# Autodesk Inventor assembly: Ensemble tout
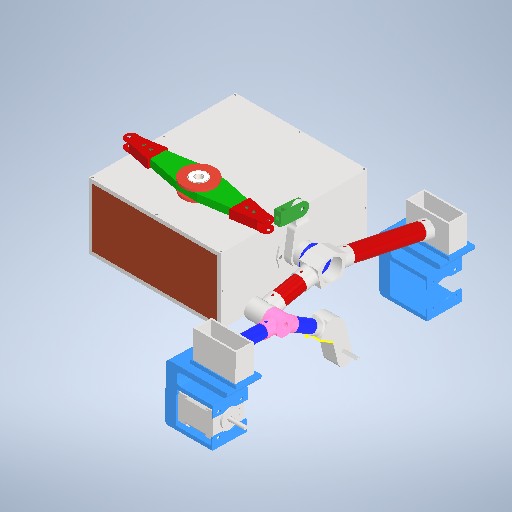
[picture p0: Inventor's stored thumbnail of the model, 512x512]
Saved by Autodesk Inventor 2026.2 (Build 302298010, 298A)
## iProperties
Created: 2026-03-16
Part Number: Ensemble tout
Document SubType Name: Assembly
Designer: genon
Author: genon
## Documents named in this file (20)
- C:\Users\genon\Documents\Henallux Passerelle\Projet de conception\Cassini T-X\Inventor\Ensemble tout.iam
- C:\Users\genon\Documents\Henallux Passerelle\Projet de conception\Cassini T-X\Inventor\Ensemble_Boite_chassis.iam
- C:\Users\genon\Documents\Henallux Passerelle\Projet de conception\Cassini T-X\Inventor\Suspension\Ensemble_Relier_suspension.iam
- C:\Users\genon\Documents\Henallux Passerelle\Projet de conception\Cassini T-X\Inventor\Suspension\tube vers bogie.ipt
- C:\Users\genon\Documents\Henallux Passerelle\Projet de conception\Cassini T-X\Inventor\Suspension\bielle sup.ipt
- C:\Users\genon\Documents\Henallux Passerelle\Projet de conception\Cassini T-X\Inventor\Suspension\bielle côté 0.ipt
- C:\Users\genon\Documents\Henallux Passerelle\Projet de conception\Cassini T-X\Inventor\Suspension\bièlle côté.ipt
- C:\Users\genon\Documents\Henallux Passerelle\Projet de conception\Cassini T-X\Inventor\Suspension\Rolling v2.ipt
- C:\Users\genon\Documents\Henallux Passerelle\Projet de conception\Cassini T-X\Inventor\Suspension\bielle côté 2.ipt
- C:\Users\genon\Documents\Henallux Passerelle\Projet de conception\Cassini T-X\Inventor\Suspension\bielle côté 3.ipt
- C:\Users\genon\Documents\Henallux Passerelle\Projet de conception\Cassini T-X\Inventor\Suspension\tubelong_rocker.ipt
- C:\Users\genon\Documents\Henallux Passerelle\Projet de conception\Cassini T-X\Inventor\Suspension\Attache servomoteur.ipt
- C:\Users\genon\Documents\Henallux Passerelle\Projet de conception\Cassini T-X\Inventor\Suspension\Attache moteur.ipt
- C:\Users\genon\Documents\Henallux Passerelle\Projet de conception\Cassini T-X\Inventor\Suspension\bielle rocker.ipt
- C:\Users\genon\Documents\Henallux Passerelle\Projet de conception\Cassini T-X\Inventor\Suspension\bielle rocker2.ipt
- C:\Users\genon\Documents\Henallux Passerelle\Projet de conception\Cassini T-X\Inventor\Suspension\tube des bogies.ipt
- C:\Users\genon\Documents\Henallux Passerelle\Projet de conception\Cassini T-X\Inventor\Suspension\bielle roue milieu.ipt
- C:\Users\genon\Documents\Henallux Passerelle\Projet de conception\Cassini T-X\Inventor\Suspension\Attache servomoteur_bogie.ipt
- C:\Users\genon\Documents\Henallux Passerelle\Projet de conception\Cassini T-X\Inventor\Suspension\mr_105_2rs.ipt
- C:\Users\genon\Downloads\nema17_17hs19-2004s1_stepperonline-1.snapshot.1\NEMA17_17HS19-2004S1_Stepperonline\NEMA17_17HS19-2004S1_Stepperonline\NEMA17_17HS19-2004S1_Stepperonline.ipt
## Components (23 placed, 19 different names)
1. Ensemble_Boite_chassis:1 [sub-assembly] — Placage:1, Placage:2, Placage:15, Placage:16, Placage:17
2. Ensemble_Relier_suspension:1 [sub-assembly] — Placage:1, Placage:2
3. bielle sup:1 — Placage:53, Placage:54
4. bielle côté 0:1 — Placage:15, Placage:16, Placage:17, Cylindrique:2, Placage:19
5. bièlle côté:1 — Cylindrique:1, Placage:18, Placage:19, Placage:20, Placage:21, Placage:22, Cylindrique:3, Cylindrique:6, Placage:52, Placage:54
6. Rolling v2:1 — Cylindrique:1, Placage:18, Cylindrique:2
7. bielle côté 2:1 — Placage:20, Placage:21, Placage:22, Placage:23, Placage:24, Placage:25, Placage:26, Placage:27
8. Rolling v2:2 — Cylindrique:3, Placage:23
9. bielle côté 3:1 — Placage:24, Placage:25, Placage:26, Placage:27, Placage:28, Placage:29, Placage:35, Placage:36
10. tubelong_rocker:1 — Placage:28, Placage:29, Placage:30, Placage:31
11. Attache servomoteur:1 — Placage:30, Placage:31, Placage:32, Placage:33, Placage:34
12. Attache moteur:2 — Placage:32, Placage:33, Placage:34
13. tube vers bogie:3 — Placage:35, Placage:36, Placage:37, Placage:38
14. bielle rocker:1 — Placage:37, Placage:38, Cylindrique:4, Placage:39, Placage:40
15. Rolling v2:3 — Cylindrique:4, Placage:39, Cylindrique:5
16. bielle rocker2:1 — Placage:40, Cylindrique:5, Placage:41, Placage:42, Placage:43, Placage:44
17. tube des bogies:1 — Placage:43, Placage:44, Placage:47, Placage:48
18. tube des bogies:2 — Placage:41, Placage:42, Placage:45, Placage:46
19. bielle roue milieu:1 — Placage:45, Placage:46
20. Attache servomoteur_bogie:1 — Placage:47, Placage:48, Placage:49, Placage:50, Placage:51
21. Attache moteur:3 — Placage:49, Placage:50, Placage:51, Placage:55, Placage:56, Placage:57
22. mr_105_2rs:1 — Cylindrique:6, Placage:52, Placage:53
23. NEMA17_17HS19-2004S1_Stepperonline:1 — Placage:55, Placage:56, Placage:57
## Relationships (51: Mate 45, CylindricalJoint 6)
- Placage:1 [Mate]: Ensemble_Boite_chassis:1 ↔ Ensemble_Relier_suspension:1
- Placage:2 [Mate]: Ensemble_Boite_chassis:1 ↔ Ensemble_Relier_suspension:1
- Placage:15 [Mate]: Ensemble_Boite_chassis:1 ↔ bielle côté 0:1
- Placage:16 [Mate]: Ensemble_Boite_chassis:1 ↔ bielle côté 0:1
- Placage:17 [Mate]: Ensemble_Boite_chassis:1 ↔ bielle côté 0:1
- Cylindrique:1: bièlle côté:1 ↔ Rolling v2:1
- Placage:18 [Mate]: bièlle côté:1 ↔ Rolling v2:1
- Cylindrique:2: bielle côté 0:1 ↔ Rolling v2:1
- Placage:19 [Mate]: bielle côté 0:1 ↔ bièlle côté:1
- Placage:20 [Mate]: bièlle côté:1 ↔ bielle côté 2:1
- Placage:21 [Mate]: bièlle côté:1 ↔ bielle côté 2:1
- Placage:22 [Mate]: bièlle côté:1 ↔ bielle côté 2:1
- Cylindrique:3: bièlle côté:1 ↔ Rolling v2:2
- Placage:23 [Mate]: bielle côté 2:1 ↔ Rolling v2:2
- Placage:24 [Mate]: bielle côté 2:1 ↔ bielle côté 3:1
- Placage:25 [Mate]: bielle côté 2:1 ↔ bielle côté 3:1
- Placage:26 [Mate]: bielle côté 2:1 ↔ bielle côté 3:1
- Placage:27 [Mate]: bielle côté 2:1 ↔ bielle côté 3:1
- Placage:28 [Mate]: bielle côté 3:1 ↔ tubelong_rocker:1
- Placage:29 [Mate]: bielle côté 3:1 ↔ tubelong_rocker:1
- Placage:30 [Mate]: tubelong_rocker:1 ↔ Attache servomoteur:1
- Placage:31 [Mate]: tubelong_rocker:1 ↔ Attache servomoteur:1
- Placage:32 [Mate]: Attache servomoteur:1 ↔ Attache moteur:2
- Placage:33 [Mate]: Attache servomoteur:1 ↔ Attache moteur:2
- Placage:34 [Mate]: Attache servomoteur:1 ↔ Attache moteur:2
- Placage:35 [Mate]: bielle côté 3:1 ↔ tube vers bogie:3
- Placage:36 [Mate]: bielle côté 3:1 ↔ tube vers bogie:3
- Placage:37 [Mate]: tube vers bogie:3 ↔ bielle rocker:1
- Placage:38 [Mate]: tube vers bogie:3 ↔ bielle rocker:1
- Cylindrique:4: bielle rocker:1 ↔ Rolling v2:3
- Placage:39 [Mate]: bielle rocker:1 ↔ Rolling v2:3
- Placage:40 [Mate]: bielle rocker:1 ↔ bielle rocker2:1
- Cylindrique:5: Rolling v2:3 ↔ bielle rocker2:1
- Placage:41 [Mate]: bielle rocker2:1 ↔ tube des bogies:2
- Placage:42 [Mate]: bielle rocker2:1 ↔ tube des bogies:2
- Placage:43 [Mate]: bielle rocker2:1 ↔ tube des bogies:1
- Placage:44 [Mate]: bielle rocker2:1 ↔ tube des bogies:1
- Placage:45 [Mate]: tube des bogies:2 ↔ bielle roue milieu:1
- Placage:46 [Mate]: tube des bogies:2 ↔ bielle roue milieu:1
- Placage:47 [Mate]: tube des bogies:1 ↔ Attache servomoteur_bogie:1
- Placage:48 [Mate]: tube des bogies:1 ↔ Attache servomoteur_bogie:1
- Placage:49 [Mate]: Attache servomoteur_bogie:1 ↔ Attache moteur:3
- Placage:50 [Mate]: Attache servomoteur_bogie:1 ↔ Attache moteur:3
- Placage:51 [Mate]: Attache servomoteur_bogie:1 ↔ Attache moteur:3
- Cylindrique:6: bièlle côté:1 ↔ mr_105_2rs:1
- Placage:52 [Mate]: bièlle côté:1 ↔ mr_105_2rs:1
- Placage:53 [Mate]: bielle sup:1 ↔ mr_105_2rs:1
- Placage:54 [Mate]: bielle sup:1 ↔ bièlle côté:1
- Placage:55 [Mate]: Attache moteur:3 ↔ NEMA17_17HS19-2004S1_Stepperonline:1
- Placage:56 [Mate]: Attache moteur:3 ↔ NEMA17_17HS19-2004S1_Stepperonline:1
- Placage:57 [Mate]: Attache moteur:3 ↔ NEMA17_17HS19-2004S1_Stepperonline:1
